# Autodesk Inventor assembly: Clamp with Piston Assembly (new)
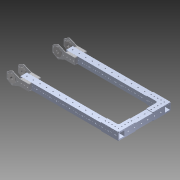
[picture p0: Inventor's stored thumbnail of the model, 180x180]
Saved by Autodesk Inventor 2014 (Build 180170000, 170)
## iProperties
Created: 2014-01-12
Part Number: Clamp with Piston Assembly (new)
Document SubType Name: Assembly
Designer: Michael
Mass: 1158.12 g
Surface Area: 2878.67 cm^2
Volume: 410.715 cm^3
Density: 2.81976 g/cm^3
Author: Michael
## Documents named in this file (7)
- C:\Users\Michael\Documents\GitHub\2014buildCAD\New Collector\Clamp with Piston Assembly (new).iam
- C:\Users\Michael\Documents\GitHub\2014buildCAD\New Collector\Vex Pro 1x1 rectangular tubing 14 in length.ipt
- C:\Users\Michael\Documents\GitHub\2014buildCAD\New Collector\Vex Pro 1x1 rectangular tubing 6 in length.ipt
- C:\Users\Michael\Documents\GitHub\2014buildCAD\New Collector\Hex Bearing 3-8 in (FR6ZZL-hex (am-0692)).ipt
- C:\Users\Michael\Documents\GitHub\2014buildCAD\New Collector\Vex Pro End Bearing Mount (Bolt).ipt
- C:\Users\Michael\Documents\GitHub\2014buildCAD\New Collector\Vex Pro 90 degree gusset.ipt
- C:\Users\Michael\Documents\GitHub\2014buildCAD\New Collector\Bearing Mount Spacer 1-8in.ipt
## Components (24 placed, 6 different names)
1. Vex Pro 1x1 rectangular tubing 14 in length:1 — Flush:1, Mate:212, Mate:220, Mate:221, Mate:222, Mate:226, Mate:227, Mate:228, Mate:243, Mate:244, Mate:245, Mate:259, Mate:262, Mate:263, Mate:264, Mate:265, Mate:266, Mate:277, Mate:278, Mate:279
2. Vex Pro 1x1 rectangular tubing 14 in length:2 — Flush:1, Mate:215, Mate:216, Mate:230, Mate:231, Mate:232, Mate:233, Mate:234, Mate:235, Mate:237, Mate:238, Mate:239, Mate:240, Mate:241, Mate:242, Mate:267, Mate:268, Mate:269, Mate:273, Mate:274, Mate:276
3. Vex Pro 1x1 rectangular tubing 6 in length:2 — Mate:223, Mate:224, Mate:225, Mate:229, Mate:236, Mate:253
4. Hex Bearing 3-8 in (FR6ZZL-hex (am-0692)):2 — Mate:201, Mate:202
5. Hex Bearing 3-8 in (FR6ZZL-hex (am-0692)):3 — Mate:203, Mate:204
6. Hex Bearing 3-8 in (FR6ZZL-hex (am-0692)):4 — Mate:179, Mate:180
7. Vex Pro End Bearing Mount (Bolt):1 — Mate:201, Mate:202, Mate:212, Mate:246, Mate:247, Mate:248
8. Vex Pro End Bearing Mount (Bolt):2 — Mate:256, Mate:257, Mate:258, Mate:260, Mate:261, Mate:263
9. Vex Pro End Bearing Mount (Bolt):3 — Mate:179, Mate:180, Mate:215, Mate:216, Mate:249, Mate:250, Mate:251
10. Vex Pro End Bearing Mount (Bolt):4 — Mate:203, Mate:204, Mate:252, Mate:254, Mate:255
11. Vex Pro 90 degree gusset:1 — Mate:220, Mate:221, Mate:222, Mate:223, Mate:224, Mate:225
12. Vex Pro 90 degree gusset:2 — Mate:226, Mate:227, Mate:228, Mate:229
13. Vex Pro 90 degree gusset:3 — Mate:230, Mate:231, Mate:232, Mate:236, Mate:253
14. Vex Pro 90 degree gusset:4 — Mate:233, Mate:234, Mate:235
15. Bearing Mount Spacer 1-8in:1 — Mate:240, Mate:241, Mate:242, Mate:252, Mate:254, Mate:255
16. Bearing Mount Spacer 1-8in:2 — Mate:237, Mate:238, Mate:239, Mate:249, Mate:250, Mate:251
17. Bearing Mount Spacer 1-8in:3 — Mate:243, Mate:244, Mate:245, Mate:246, Mate:247, Mate:248
18. Bearing Mount Spacer 1-8in:4 — Mate:256, Mate:257, Mate:258, Mate:259, Mate:262
19. Hex Bearing 3-8 in (FR6ZZL-hex (am-0692)):5 — Mate:260, Mate:261
20. Vex Pro 1x1 rectangular tubing 6 in length:3 — Mate:270, Mate:271, Mate:272, Mate:275, Mate:280
21. Vex Pro 90 degree gusset:5 — Mate:264, Mate:265, Mate:266, Mate:270, Mate:271
22. Vex Pro 90 degree gusset:6 — Mate:267, Mate:268, Mate:269, Mate:272
23. Vex Pro 90 degree gusset:7 — Mate:273, Mate:274, Mate:275, Mate:276
24. Vex Pro 90 degree gusset:8 — Mate:277, Mate:278, Mate:279, Mate:280
## Relationships (71: Mate 70, Flush 1)
- Mate:179: Hex Bearing 3-8 in (FR6ZZL-hex (am-0692)):4 ↔ Vex Pro End Bearing Mount (Bolt):3
- Mate:180: Hex Bearing 3-8 in (FR6ZZL-hex (am-0692)):4 ↔ Vex Pro End Bearing Mount (Bolt):3
- Flush:1: Vex Pro 1x1 rectangular tubing 14 in length:1 ↔ Vex Pro 1x1 rectangular tubing 14 in length:2
- Mate:201: Hex Bearing 3-8 in (FR6ZZL-hex (am-0692)):2 ↔ Vex Pro End Bearing Mount (Bolt):1
- Mate:202: Hex Bearing 3-8 in (FR6ZZL-hex (am-0692)):2 ↔ Vex Pro End Bearing Mount (Bolt):1
- Mate:203: Hex Bearing 3-8 in (FR6ZZL-hex (am-0692)):3 ↔ Vex Pro End Bearing Mount (Bolt):4
- Mate:204: Hex Bearing 3-8 in (FR6ZZL-hex (am-0692)):3 ↔ Vex Pro End Bearing Mount (Bolt):4
- Mate:212: Vex Pro 1x1 rectangular tubing 14 in length:1 ↔ Vex Pro End Bearing Mount (Bolt):1
- Mate:215: Vex Pro 1x1 rectangular tubing 14 in length:2 ↔ Vex Pro End Bearing Mount (Bolt):3
- Mate:216: Vex Pro 1x1 rectangular tubing 14 in length:2 ↔ Vex Pro End Bearing Mount (Bolt):3
- Mate:220: Vex Pro 1x1 rectangular tubing 14 in length:1 ↔ Vex Pro 90 degree gusset:1
- Mate:221: Vex Pro 1x1 rectangular tubing 14 in length:1 ↔ Vex Pro 90 degree gusset:1
- Mate:222: Vex Pro 1x1 rectangular tubing 14 in length:1 ↔ Vex Pro 90 degree gusset:1
- Mate:223: Vex Pro 1x1 rectangular tubing 6 in length:2 ↔ Vex Pro 90 degree gusset:1
- Mate:224: Vex Pro 1x1 rectangular tubing 6 in length:2 ↔ Vex Pro 90 degree gusset:1
- Mate:225: Vex Pro 1x1 rectangular tubing 6 in length:2 ↔ Vex Pro 90 degree gusset:1
- Mate:226: Vex Pro 1x1 rectangular tubing 14 in length:1 ↔ Vex Pro 90 degree gusset:2
- Mate:227: Vex Pro 1x1 rectangular tubing 14 in length:1 ↔ Vex Pro 90 degree gusset:2
- Mate:228: Vex Pro 1x1 rectangular tubing 14 in length:1 ↔ Vex Pro 90 degree gusset:2
- Mate:229: Vex Pro 1x1 rectangular tubing 6 in length:2 ↔ Vex Pro 90 degree gusset:2
- Mate:230: Vex Pro 1x1 rectangular tubing 14 in length:2 ↔ Vex Pro 90 degree gusset:3
- Mate:231: Vex Pro 1x1 rectangular tubing 14 in length:2 ↔ Vex Pro 90 degree gusset:3
- Mate:232: Vex Pro 1x1 rectangular tubing 14 in length:2 ↔ Vex Pro 90 degree gusset:3
- Mate:233: Vex Pro 1x1 rectangular tubing 14 in length:2 ↔ Vex Pro 90 degree gusset:4
- Mate:234: Vex Pro 1x1 rectangular tubing 14 in length:2 ↔ Vex Pro 90 degree gusset:4
- Mate:235: Vex Pro 1x1 rectangular tubing 14 in length:2 ↔ Vex Pro 90 degree gusset:4
- Mate:236: Vex Pro 1x1 rectangular tubing 6 in length:2 ↔ Vex Pro 90 degree gusset:3
- Mate:237: Vex Pro 1x1 rectangular tubing 14 in length:2 ↔ Bearing Mount Spacer 1-8in:2
- Mate:238: Vex Pro 1x1 rectangular tubing 14 in length:2 ↔ Bearing Mount Spacer 1-8in:2
- Mate:239: Vex Pro 1x1 rectangular tubing 14 in length:2 ↔ Bearing Mount Spacer 1-8in:2
- Mate:240: Vex Pro 1x1 rectangular tubing 14 in length:2 ↔ Bearing Mount Spacer 1-8in:1
- Mate:241: Vex Pro 1x1 rectangular tubing 14 in length:2 ↔ Bearing Mount Spacer 1-8in:1
- Mate:242: Vex Pro 1x1 rectangular tubing 14 in length:2 ↔ Bearing Mount Spacer 1-8in:1
- Mate:243: Vex Pro 1x1 rectangular tubing 14 in length:1 ↔ Bearing Mount Spacer 1-8in:3
- Mate:244: Vex Pro 1x1 rectangular tubing 14 in length:1 ↔ Bearing Mount Spacer 1-8in:3
- Mate:245: Vex Pro 1x1 rectangular tubing 14 in length:1 ↔ Bearing Mount Spacer 1-8in:3
- Mate:246: Vex Pro End Bearing Mount (Bolt):1 ↔ Bearing Mount Spacer 1-8in:3
- Mate:247: Vex Pro End Bearing Mount (Bolt):1 ↔ Bearing Mount Spacer 1-8in:3
- Mate:248: Vex Pro End Bearing Mount (Bolt):1 ↔ Bearing Mount Spacer 1-8in:3
- Mate:249: Vex Pro End Bearing Mount (Bolt):3 ↔ Bearing Mount Spacer 1-8in:2
- Mate:250: Vex Pro End Bearing Mount (Bolt):3 ↔ Bearing Mount Spacer 1-8in:2
- Mate:251: Vex Pro End Bearing Mount (Bolt):3 ↔ Bearing Mount Spacer 1-8in:2
- Mate:252: Vex Pro End Bearing Mount (Bolt):4 ↔ Bearing Mount Spacer 1-8in:1
- Mate:253: Vex Pro 1x1 rectangular tubing 6 in length:2 ↔ Vex Pro 90 degree gusset:3
- Mate:254: Vex Pro End Bearing Mount (Bolt):4 ↔ Bearing Mount Spacer 1-8in:1
- Mate:255: Vex Pro End Bearing Mount (Bolt):4 ↔ Bearing Mount Spacer 1-8in:1
- Mate:256: Vex Pro End Bearing Mount (Bolt):2 ↔ Bearing Mount Spacer 1-8in:4
- Mate:257: Vex Pro End Bearing Mount (Bolt):2 ↔ Bearing Mount Spacer 1-8in:4
- Mate:258: Vex Pro End Bearing Mount (Bolt):2 ↔ Bearing Mount Spacer 1-8in:4
- Mate:259: Vex Pro 1x1 rectangular tubing 14 in length:1 ↔ Bearing Mount Spacer 1-8in:4
- Mate:260: Vex Pro End Bearing Mount (Bolt):2 ↔ Hex Bearing 3-8 in (FR6ZZL-hex (am-0692)):5
- Mate:261: Vex Pro End Bearing Mount (Bolt):2 ↔ Hex Bearing 3-8 in (FR6ZZL-hex (am-0692)):5
- Mate:262: Vex Pro 1x1 rectangular tubing 14 in length:1 ↔ Bearing Mount Spacer 1-8in:4
- Mate:263: Vex Pro 1x1 rectangular tubing 14 in length:1 ↔ Vex Pro End Bearing Mount (Bolt):2
- Mate:264: Vex Pro 1x1 rectangular tubing 14 in length:1 ↔ Vex Pro 90 degree gusset:5
- Mate:265: Vex Pro 1x1 rectangular tubing 14 in length:1 ↔ Vex Pro 90 degree gusset:5
- Mate:266: Vex Pro 1x1 rectangular tubing 14 in length:1 ↔ Vex Pro 90 degree gusset:5
- Mate:267: Vex Pro 1x1 rectangular tubing 14 in length:2 ↔ Vex Pro 90 degree gusset:6
- Mate:268: Vex Pro 1x1 rectangular tubing 14 in length:2 ↔ Vex Pro 90 degree gusset:6
- Mate:269: Vex Pro 1x1 rectangular tubing 14 in length:2 ↔ Vex Pro 90 degree gusset:6
- Mate:270: Vex Pro 1x1 rectangular tubing 6 in length:3 ↔ Vex Pro 90 degree gusset:5
- Mate:271: Vex Pro 1x1 rectangular tubing 6 in length:3 ↔ Vex Pro 90 degree gusset:5
- Mate:272: Vex Pro 1x1 rectangular tubing 6 in length:3 ↔ Vex Pro 90 degree gusset:6
- Mate:273: Vex Pro 1x1 rectangular tubing 14 in length:2 ↔ Vex Pro 90 degree gusset:7
- Mate:274: Vex Pro 1x1 rectangular tubing 14 in length:2 ↔ Vex Pro 90 degree gusset:7
- Mate:275: Vex Pro 1x1 rectangular tubing 6 in length:3 ↔ Vex Pro 90 degree gusset:7
- Mate:276: Vex Pro 1x1 rectangular tubing 14 in length:2 ↔ Vex Pro 90 degree gusset:7
- Mate:277: Vex Pro 1x1 rectangular tubing 14 in length:1 ↔ Vex Pro 90 degree gusset:8
- Mate:278: Vex Pro 1x1 rectangular tubing 14 in length:1 ↔ Vex Pro 90 degree gusset:8
- Mate:279: Vex Pro 1x1 rectangular tubing 14 in length:1 ↔ Vex Pro 90 degree gusset:8
- Mate:280: Vex Pro 1x1 rectangular tubing 6 in length:3 ↔ Vex Pro 90 degree gusset:8
